# Autodesk Inventor assembly: FULL BOX
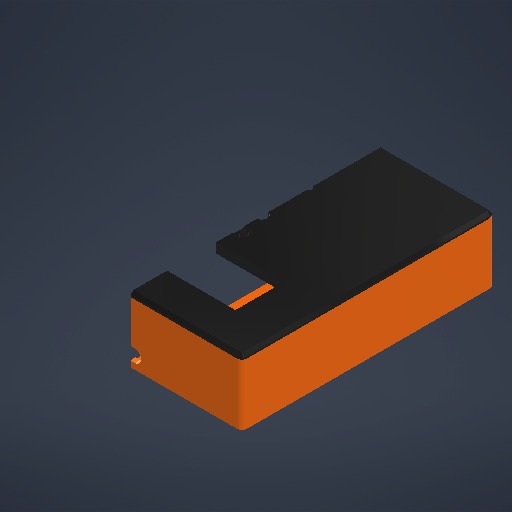
[picture p0: Inventor's stored thumbnail of the model, 512x512]
Saved by Autodesk Inventor 2026 (Build 300175000, 175)
## iProperties
Created: 2025-06-07
Part Number: FULL BOX
Document SubType Name: Assembly
Designer: asus
Author: asus
## Documents named in this file (3)
- C:\Users\asus\OneDrive\Documents\Projects\TRACKING DEVICE\FULL BOX.iam
- C:\Users\asus\OneDrive\Documents\Projects\TRACKING DEVICE\LID_FINAL.ipt
- C:\Users\asus\OneDrive\Documents\Projects\TRACKING DEVICE\BOX.ipt
## Components (2 placed, 2 different names)
1. LID_FINAL:1 — Mate:1, Flush:1, Flush:2, Flush:3, Flush:4
2. BOX:1 — Mate:1, Flush:1, Flush:2, Flush:3, Flush:4
## Relationships (5: Flush 4, Mate 1)
- Mate:1: LID_FINAL:1 ↔ BOX:1
- Flush:1: LID_FINAL:1 ↔ BOX:1
- Flush:2: LID_FINAL:1 ↔ BOX:1
- Flush:3: LID_FINAL:1 ↔ BOX:1
- Flush:4: LID_FINAL:1 ↔ BOX:1
